# Autodesk Inventor assembly: front_box
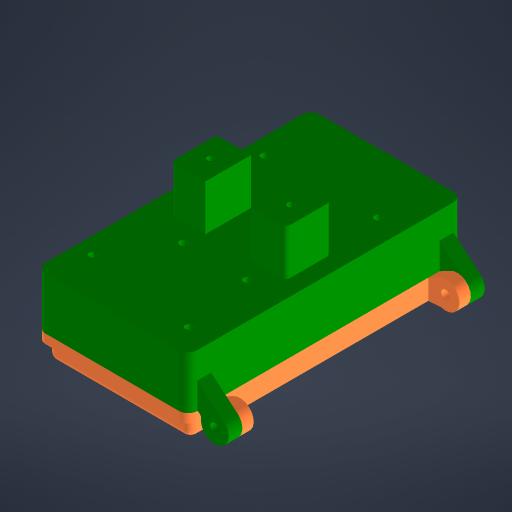
[picture p0: Inventor's stored thumbnail of the model, 512x512]
Saved by Autodesk Inventor 2024 (Build 280153000, 153)
## iProperties
Created: 2023-05-12
Part Number: front_box
Document SubType Name: Assembly
Designer: user
Author: user
## Documents named in this file (3)
- D:\Docs\Robot\3d\machine_body\front_box.iam
- D:\Docs\Robot\3d\machine_body\front_box\front_box.ipt
- D:\Docs\Robot\3d\machine_body\front_box\front_box_cup.ipt
## Components (2 placed, 2 different names)
1. front_box:1 — Совмещение:1, Заподлицо:1, Совмещение:2, Вставка:1
2. front_box_cup:1 — Вставка:1
## Relationships (4: Mate 2, Flush 1, Insert 1)
- Совмещение:1 [Mate]: front_box:1
- Заподлицо:1 [Flush]: front_box:1
- Совмещение:2 [Mate]: front_box:1
- Вставка:1 [Insert]: front_box:1 ↔ front_box_cup:1
